# Autodesk Inventor assembly: Kit Frame 24x32
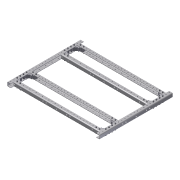
[picture p0: Inventor's stored thumbnail of the model, 180x180]
Saved by Autodesk Inventor 2013 (Build 170138000, 138)
## iProperties
Created: 2013-01-06
Part Number: Kit Frame 24x32
Document SubType Name: Assembly
Designer: Nemo
Author: Nemo
## Documents named in this file (4)
- H:\Nemo\Documents\Robotics\COTS Parts\Kit Frame - AndyMark\Kit Frame 22x34.iam
- H:\Nemo\Documents\Robotics\COTS Parts\Kit Frame - AndyMark\Components\22x34 Side Rail sub.iam
- H:\Nemo\Documents\Robotics\COTS Parts\Kit Frame - AndyMark\Components\22x34 Side Rail Sub mirror.iam
- H:\Nemo\Documents\Robotics\COTS Parts\Kit Frame - AndyMark\Components\C Channel - FrontBack 22x34.ipt
## Components (6 placed, 3 different names)
1. C Channel - Cut-01:3 — Flush:5
2. C Channel - Cut-01:4 — Mate:3, Insert:6, Mate:12, Mate:13, Insert:7, Mate:14, Insert:8
3. 22x34 Side Rail sub:1 [sub-assembly] — Mate:13
4. 22x34 Side Rail sub:2 [sub-assembly] — Insert:7, Mate:14
5. 22x34 Side Rail Sub mirror:2 [sub-assembly] — Insert:8
6. 22x34 Side Rail Sub mirror:1 [sub-assembly] — Insert:6, Mate:12
## Relationships (14: Mate 6, Flush 5, Insert 3)
- [Mate] (36.83 mm): 22x34 Side Rail sub:1
- [Flush]: 22x34 Side Rail sub:1 ↔ 22x34 Side Rail Sub mirror:2
- [Mate]: 22x34 Side Rail sub:1
- [Flush]: 22x34 Side Rail Sub mirror:2
- [Flush]: C Channel - Cut-01:3 ↔ 22x34 Side Rail sub:1
- [Flush]: C Channel - Cut-01:4 ↔ 22x34 Side Rail sub:1
- Flush:5: C Channel - Cut-01:3
- Mate:3: C Channel - Cut-01:4
- Insert:6: C Channel - Cut-01:4 ↔ 22x34 Side Rail Sub mirror:1
- Mate:12: C Channel - Cut-01:4 ↔ 22x34 Side Rail Sub mirror:1
- Mate:13: C Channel - Cut-01:4 ↔ 22x34 Side Rail sub:1
- Insert:7: C Channel - Cut-01:4 ↔ 22x34 Side Rail sub:2
- Mate:14: C Channel - Cut-01:4 ↔ 22x34 Side Rail sub:2
- Insert:8: C Channel - Cut-01:4 ↔ 22x34 Side Rail Sub mirror:2
